# Autodesk Inventor assembly: крепление шестерни
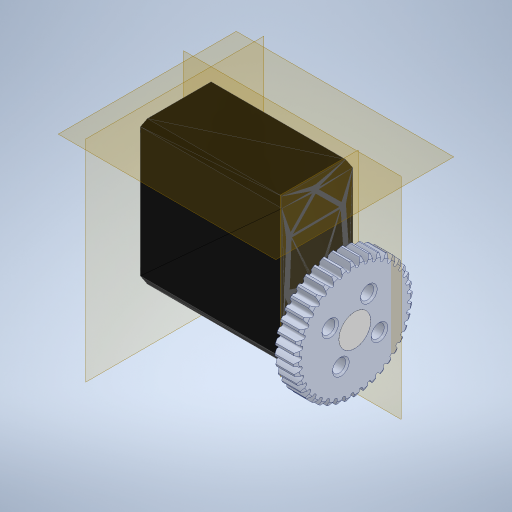
[picture p0: Inventor's stored thumbnail of the model, 512x512]
Saved by Autodesk Inventor 2023.1 (Build 271208000, 208)
## iProperties
Created: 2024-12-03
Part Number: крепление шестерни
Document SubType Name: Assembly
Designer: DELL
Author: DELL
## Documents named in this file (4)
- C:\Users\DELL\Desktop\Cheburashka_construction\Cheburashka\cheb\крепление шестерни.iam
- C:\Users\DELL\Desktop\Cheburashka_construction\Cheburashka\cheb\Импорт\Servo.ipt
- C:\Users\DELL\Desktop\Cheburashka_construction\Cheburashka\cheb\Импорт\Pitsco Education-739028.ipt
- C:\Users\DELL\Desktop\Cheburashka_construction\Cheburashka\cheb\Деталь2.ipt
## Components (3 placed, 3 different names)
1. Servo:1 — Совмещение:1, Совмещение:2, Совмещение:3, Заподлицо:1, Совмещение:4, Угол:1
2. Pitsco Education-739028:1 — Совмещение:1, Совмещение:5
3. Деталь2:1 — Заподлицо:2, Совмещение:5
## Relationships (8: Mate 5, Flush 2, Angle 1)
- Совмещение:1 [Mate]: Servo:1 ↔ Pitsco Education-739028:1
- Совмещение:2 [Mate]: Servo:1
- Совмещение:3 [Mate]: Servo:1
- Заподлицо:1 [Flush]: Servo:1
- Совмещение:4 [Mate]: Servo:1
- Угол:1 [Angle] (0 deg): Servo:1
- Заподлицо:2 [Flush]: Деталь2:1
- Совмещение:5 [Mate]: Pitsco Education-739028:1 ↔ Деталь2:1
